# Autodesk Inventor assembly: BodyStructure
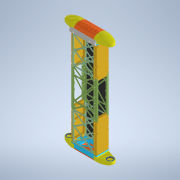
[picture p0: Inventor's stored thumbnail of the model, 180x180]
Saved by Autodesk Inventor 2022.2 (Build 262287030, 287C)
## iProperties
Created: 2022-01-14
Part Number: BodyStructure
Document SubType Name: Assembly
Designer: Jochen
Author: Jochen
## Documents named in this file (10)
- D:\Projects\Lisbeth\CAD\BodyStructure.iam
- D:\Projects\Lisbeth\CAD\Body\BodyStructure Side.ipt
- D:\Projects\Lisbeth\CAD\Body\BodyStructure HipSupport.ipt
- D:\Projects\Lisbeth\CAD\Body\BodyStructure Front.ipt
- D:\Projects\Lisbeth\CAD\Body\BodyStructure Centre.ipt
- D:\Projects\Lisbeth\CAD\Body\BodyStructure Plate.ipt
- D:\Projects\Lisbeth\CAD\Common\Bearing\bearing_27_20_4 s61704-2rsr.ipt
- D:\Projects\Lisbeth\CAD\Body\BodyCover.ipt
- D:\Projects\Lisbeth\CAD\Common\Battery\Battery Pack.ipt
- D:\Projects\Lisbeth\CAD\Body\BodyDampener.ipt
## Components (25 placed, 8 different names)
1. BodyStructure Side:1 — Mate:9, Flush:1, Mate:11, Mate:49, Mate:50, Mate:55, Mate:65, Mate:73, Mate:75
2. BodyStructure Side:2 — Mate:51, Mate:52, Mate:53, Mate:56, Mate:66, Mate:74
3. BodyHipSupport:1 — Mate:38, Mate:39, Mate:76, Mate:77
4. BodyHipSupport:2 — Mate:44, Mate:45, Mate:78, Mate:79
5. Body Structure Centre:1 — Mate:9, Flush:1, Mate:13, Mate:14, Mate:15, Mate:16, Mate:51, Mate:59
6. Body Structure Centre:2 — Mate:11, Mate:46, Mate:49, Mate:52
7. BodyStructure Side:3 — Mate:13, Mate:16, Mate:20, Mate:28, Mate:46, Mate:48, Mate:63
8. BodyStructure Side:4 — Mate:14, Mate:15, Mate:19, Mate:57, Mate:58
9. BodyStructure Front:2 — Mate:19, Mate:20, Mate:21, Mate:22, Mate:23, Mate:24, Mate:64, 0, Mate:69, Mate:70, Mate:71, Mate:72
10. BodyHipSupport:3 — Mate:23, Mate:24, Mate:42, Mate:43
11. BodyHipSupport:4 — Mate:21, Mate:22, Mate:40, Mate:41
12. Body Structure Centre:3 — Mate:53, Mate:55, Mate:56
13. Body Structure Centre:4 — Mate:28, Mate:58, Mate:60, Mate:61
14. Body Structure Centre:5 — Mate:50, Mate:65, Mate:66
15. Body Structure Centre:6 — Mate:48, Mate:57, Mate:63
16. bearing_27_20_4 s61704-2rsr:1 — Mate:38, Mate:39
17. bearing_27_20_4 s61704-2rsr:2 — Mate:44, Mate:45
18. bearing_27_20_4 s61704-2rsr:3 — Mate:40, Mate:41
19. bearing_27_20_4 s61704-2rsr:4 — Mate:42, Mate:43
20. BodyCover:1 — Mate:59, Mate:60, Mate:61
21. BodyCover:2 — Mate:64
22. Battery Pack 59x31x21:1
23. BodySiliconeRubber:1 — 0, Mate:69, Mate:70
24. BodySiliconeRubber:2 — Mate:71, Mate:72
25. BodyStructure Front:3 — Mate:73, Mate:74, Mate:75, Mate:76, Mate:77, Mate:78, Mate:79
## Relationships (52: Mate 50, Flush 2)
- Mate:9: BodyStructure Side:1 ↔ Body Structure Centre:1
- Flush:1: BodyStructure Side:1 ↔ Body Structure Centre:1
- Mate:11: BodyStructure Side:1 ↔ Body Structure Centre:2
- Mate:13: Body Structure Centre:1 ↔ BodyStructure Side:3
- Mate:14: Body Structure Centre:1 ↔ BodyStructure Side:4
- Mate:15: Body Structure Centre:1 ↔ BodyStructure Side:4
- Mate:16: Body Structure Centre:1 ↔ BodyStructure Side:3
- Mate:19: BodyStructure Side:4 ↔ BodyStructure Front:2
- Mate:20: BodyStructure Side:3 ↔ BodyStructure Front:2
- Mate:21: BodyStructure Front:2 ↔ BodyHipSupport:4
- Mate:22: BodyStructure Front:2 ↔ BodyHipSupport:4
- Mate:23: BodyStructure Front:2 ↔ BodyHipSupport:3
- Mate:24: BodyStructure Front:2 ↔ BodyHipSupport:3
- Mate:28: BodyStructure Side:3 ↔ Body Structure Centre:4
- Mate:38: BodyHipSupport:1 ↔ bearing_27_20_4 s61704-2rsr:1
- Mate:39: BodyHipSupport:1 ↔ bearing_27_20_4 s61704-2rsr:1
- Mate:40: BodyHipSupport:4 ↔ bearing_27_20_4 s61704-2rsr:3
- Mate:41: BodyHipSupport:4 ↔ bearing_27_20_4 s61704-2rsr:3
- Mate:42: BodyHipSupport:3 ↔ bearing_27_20_4 s61704-2rsr:4
- Mate:43: BodyHipSupport:3 ↔ bearing_27_20_4 s61704-2rsr:4
- Mate:44: BodyHipSupport:2 ↔ bearing_27_20_4 s61704-2rsr:2
- Mate:45: BodyHipSupport:2 ↔ bearing_27_20_4 s61704-2rsr:2
- Mate:46: Body Structure Centre:2 ↔ BodyStructure Side:3
- Mate:48: BodyStructure Side:3 ↔ Body Structure Centre:6
- Mate:49: BodyStructure Side:1 ↔ Body Structure Centre:2
- Mate:50: BodyStructure Side:1 ↔ Body Structure Centre:5
- Mate:51: BodyStructure Side:2 ↔ Body Structure Centre:1
- Mate:52: BodyStructure Side:2 ↔ Body Structure Centre:2
- Mate:53: BodyStructure Side:2 ↔ Body Structure Centre:3
- Mate:55: BodyStructure Side:1 ↔ Body Structure Centre:3
- Mate:56: BodyStructure Side:2 ↔ Body Structure Centre:3
- Mate:57: BodyStructure Side:4 ↔ Body Structure Centre:6
- Mate:58: BodyStructure Side:4 ↔ Body Structure Centre:4
- Mate:59: Body Structure Centre:1 ↔ BodyCover:1
- Mate:60: Body Structure Centre:4 ↔ BodyCover:1
- Mate:61: Body Structure Centre:4 ↔ BodyCover:1
- Mate:63: BodyStructure Side:3 ↔ Body Structure Centre:6
- Mate:64: BodyStructure Front:2 ↔ BodyCover:2
- Mate:65: BodyStructure Side:1 ↔ Body Structure Centre:5
- Mate:66: BodyStructure Side:2 ↔ Body Structure Centre:5
- 0 [Flush] (12.5 mm): BodyStructure Front:2 ↔ BodySiliconeRubber:1
- Mate:69: BodyStructure Front:2 ↔ BodySiliconeRubber:1
- Mate:70: BodyStructure Front:2 ↔ BodySiliconeRubber:1
- Mate:71: BodyStructure Front:2 ↔ BodySiliconeRubber:2
- Mate:72: BodyStructure Front:2 ↔ BodySiliconeRubber:2
- Mate:73: BodyStructure Side:1 ↔ BodyStructure Front:3
- Mate:74: BodyStructure Side:2 ↔ BodyStructure Front:3
- Mate:75: BodyStructure Side:1 ↔ BodyStructure Front:3
- Mate:76: BodyHipSupport:1 ↔ BodyStructure Front:3
- Mate:77: BodyHipSupport:1 ↔ BodyStructure Front:3
- Mate:78: BodyHipSupport:2 ↔ BodyStructure Front:3
- Mate:79: BodyHipSupport:2 ↔ BodyStructure Front:3
